# Autodesk Inventor assembly: motor with bevil gear and sprocket
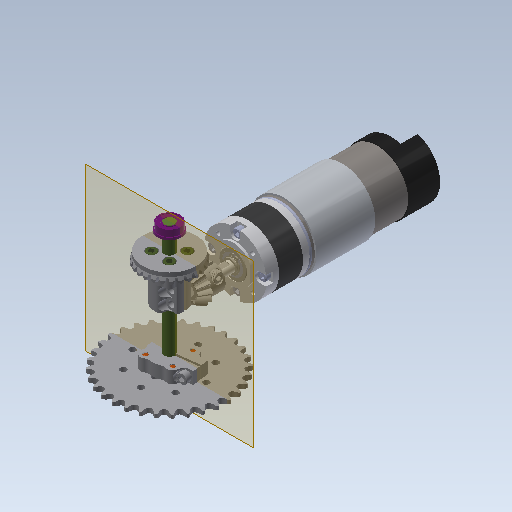
[picture p0: Inventor's stored thumbnail of the model, 512x512]
Saved by Autodesk Inventor 2020 (Build 240168000, 168)
## iProperties
Created: 2019-09-29
Part Number: motor with bevil gear and sprocket
Document SubType Name: Assembly
Designer: ball
Author: ball
## Documents named in this file (3)
- D:\FTC8863\2019 Robot\Mecanum Drive Train\motor with bevil gear and sprocket.iam
- D:\FTC8863\2019 Robot\Mecanum Drive Train\motor with bevel pinion gear.iam
- D:\FTC8863\2019 Robot\Mecanum Drive Train\sprocket and bevel gear on shaft.iam
## Components (2 placed, 2 different names)
1. motor with bevel pinion gear:1 [sub-assembly] — Flush:1, Flush:2, Flush:3, Flush:4
2. sprocket and bevel gear on shaft:1 [sub-assembly] — Flush:1, Flush:2, Flush:3, Flush:4
## Relationships (4: Flush 4)
- Flush:1: motor with bevel pinion gear:1 ↔ sprocket and bevel gear on shaft:1
- Flush:2: motor with bevel pinion gear:1 ↔ sprocket and bevel gear on shaft:1
- Flush:3 (-11.176 mm): motor with bevel pinion gear:1 ↔ sprocket and bevel gear on shaft:1
- Flush:4 (-12.7 mm): motor with bevel pinion gear:1 ↔ sprocket and bevel gear on shaft:1
